# Autodesk Inventor assembly: Abstandslehre#
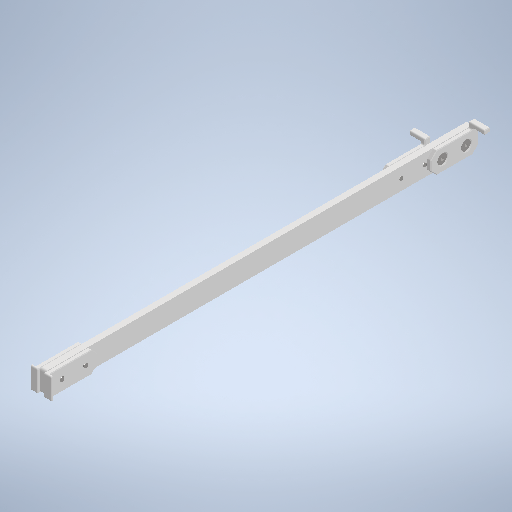
[picture p0: Inventor's stored thumbnail of the model, 512x512]
Saved by Autodesk Inventor 2025.1 (Build 291241000, 241)
## iProperties
Created: 2024-11-26
Part Number: Abstandslehre#
Document SubType Name: Assembly
Designer: Kai Altwicker
Author: Kai Altwicker
## Documents named in this file (8)
- C:\Users\tallA\Repos\VolumanXR\hardware-capture\cad\rig_v2\Abstandslehre\Abstandslehre#.iam
- C:\Users\tallA\Repos\VolumanXR\hardware-capture\cad\rig_v2\Abstandslehre\Sstab.ipt
- C:\Users\tallA\Repos\VolumanXR\hardware-capture\cad\rig_v2\Abstandslehre\Fuß.ipt
- C:\Users\tallA\Repos\VolumanXR\hardware-capture\cad\rig_v2\Abstandslehre\Kopf.ipt
- C:\Users\tallA\Repos\VolumanXR\hardware-capture\cad\rig_v2\Abstandslehre\Kopf_MIR.ipt
- Z:\WINDOWS\Documents\Inventor\Content Center Files\R2025\de-DE\DIN 7991(2)\DIN 7991 - M4x8.ipt
- Z:\WINDOWS\Documents\Inventor\Content Center Files\R2025\de-DE\DIN 7991(2)\DIN 7991 - M4x12.ipt
- C:\Users\tallA\Repos\VolumanXR\hardware-capture\cad\dimensions.xlsx
## Components (10 placed, 6 different names)
1. Sstab:1 — Passend:1, Passend:2, Passend:3, Passend:4, Passend:5, Passend:6
2. Fuß:1 — Passend:5, Passend:6, Passend:9, Passend:10
3. Kopf:1 — Passend:3, Passend:4, Passend:7, Passend:8
4. Kopf_MIR:1 — Passend:1, Passend:2, Passend:11, Passend:12
5. DIN 7991 M4x8:1 — Passend:7
6. DIN 7991 M4x8:2 — Passend:8
7. DIN 7991 M4x12:1 — Passend:9
8. DIN 7991 M4x12:2 — Passend:10
9. DIN 7991 M4x8:5 — Passend:11
10. DIN 7991 M4x8:6 — Passend:12
## Relationships (12: Mate 12)
- Passend:1 [Mate]: Sstab:1 ↔ Kopf_MIR:1
- Passend:2 [Mate]: Sstab:1 ↔ Kopf_MIR:1
- Passend:3 [Mate]: Sstab:1 ↔ Kopf:1
- Passend:4 [Mate]: Sstab:1 ↔ Kopf:1
- Passend:5 [Mate]: Sstab:1 ↔ Fuß:1
- Passend:6 [Mate]: Sstab:1 ↔ Fuß:1
- Passend:7 [Mate]: Kopf:1 ↔ DIN 7991 M4x8:1
- Passend:8 [Mate]: Kopf:1 ↔ DIN 7991 M4x8:2
- Passend:9 [Mate]: Fuß:1 ↔ DIN 7991 M4x12:1
- Passend:10 [Mate]: Fuß:1 ↔ DIN 7991 M4x12:2
- Passend:11 [Mate]: Kopf_MIR:1 ↔ DIN 7991 M4x8:5
- Passend:12 [Mate]: Kopf_MIR:1 ↔ DIN 7991 M4x8:6
## Named parameters: d_tol = 0.3 mm, d_wand = 1.5 mm, l_profil_traeger = 1500 mm, l_profil_staender = 2500 mm, h_profil_40x40 = 40 mm, b_profil_40x40 = 40 mm, h_profil_20x20 = 20 mm, b_profil_20x20 = 20 mm, b_rasp_pi = 56 mm, w_kamera_hori = 66 deg, r_rasp_pi = 3 mm, l_rasp_pi = 85 mm, D_oct = 3621.32034 mm, D_hexadeca = 7541.00924 mm, w_kamera_vert = 41 deg, d_traeger = 625 mm, l_profil_40x40 = 2500 mm, l_profil_20x20 = 1500 mm
